# Autodesk Inventor assembly: Full_Assembly_2_0_2
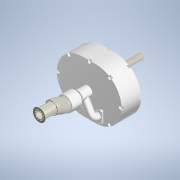
[picture p0: Inventor's stored thumbnail of the model, 180x180]
Saved by Autodesk Inventor 2021 (Build 250183000, 183)
## iProperties
Created: 2021-04-14
Part Number: Full_Assembly_2_0_2
Document SubType Name: Assembly
Designer: lucia
Mass: 12850.4 g
Surface Area: 5748.06 cm^2
Volume: 2623.18 cm^3
Density: 4.89877 g/cm^3
Author: lucia
## Documents named in this file (10)
- E:\Documents\Inventor\Fixed Rotor Wankel Engine\Assemblies\Full_Assembly_2_0_2.iam
- E:\Documents\Inventor\Fixed Rotor Wankel Engine\Parts\Rotor_Mount.ipt
- E:\Documents\Inventor\Fixed Rotor Wankel Engine\Parts\Eccentric_Shaft_2.ipt
- E:\Documents\Inventor\Fixed Rotor Wankel Engine\Parts\Rotor_Geared_6t_Mountable.ipt
- E:\Documents\Inventor\Fixed Rotor Wankel Engine\Parts\Side_Plate_Combined_Intake_Exhaust.ipt
- E:\Documents\Inventor\Fixed Rotor Wankel Engine\Parts\Housing.ipt
- E:\Documents\Inventor\Fixed Rotor Wankel Engine\Parts\Side_Plate_Blank.ipt
- E:\Documents\Inventor\Fixed Rotor Wankel Engine\Parts\Combined_Intake_Exhaust_Manifold.ipt
- E:\Documents\Inventor\Fixed Rotor Wankel Engine\Parts\Intake_Manifold_2.ipt
- E:\Documents\Inventor\Fixed Rotor Wankel Engine\Parts\Exhaust_Manifold_2_2.ipt
## Components (9 placed, 9 different names)
1. Rotor_Mount:1 — Mate:1, Mate:2, Mate:3, Mate:4, Mate:5, Mate:6, Mate:7
2. Eccentric_Shaft_2:1 — Mate:3, Mate:4, Mate:9, Mate:16, Mate:17, Mate:18, Mate:Correct_Position, Rotation:1
3. Rotor_Geared_6t_Mountable:1 — Mate:5, Mate:6, Mate:7, Mate:8
4. Side_Plate_Combined_Intake_Exhaust:1 — Mate:8, Mate:9, Mate:10, Mate:11, Mate:12, Mate:Correct_Position_2, Rotation:1, Mate:27, Mate:28, Mate:26, Mate:29, Mate:30, Mate:31
5. Housing:1 — Mate:10, Mate:11, Mate:12, Mate:13, Mate:14, Mate:15
6. Side_Plate_Blank:1 — Mate:13, Mate:14, Mate:15
7. Combined_Intake_Exhaust_Manifold:1 — Mate:16, Mate:17, Mate:18
8. Intake_Manifold_2:1 — Mate:27, Mate:28, Mate:26
9. Exhaust_Manifold_2_2:1 — Mate:29, Mate:30, Mate:31
## Relationships (27: Mate 26, RelateRotation 1)
- Mate:1: Rotor_Mount:1
- Mate:2: Rotor_Mount:1
- Mate:3: Rotor_Mount:1 ↔ Eccentric_Shaft_2:1
- Mate:4: Rotor_Mount:1 ↔ Eccentric_Shaft_2:1
- Mate:5: Rotor_Mount:1 ↔ Rotor_Geared_6t_Mountable:1
- Mate:6: Rotor_Mount:1 ↔ Rotor_Geared_6t_Mountable:1
- Mate:7: Rotor_Mount:1 ↔ Rotor_Geared_6t_Mountable:1
- Mate:8: Rotor_Geared_6t_Mountable:1 ↔ Side_Plate_Combined_Intake_Exhaust:1
- Mate:9: Eccentric_Shaft_2:1 ↔ Side_Plate_Combined_Intake_Exhaust:1
- Mate:10: Side_Plate_Combined_Intake_Exhaust:1 ↔ Housing:1
- Mate:11: Side_Plate_Combined_Intake_Exhaust:1 ↔ Housing:1
- Mate:12: Side_Plate_Combined_Intake_Exhaust:1 ↔ Housing:1
- Mate:13: Housing:1 ↔ Side_Plate_Blank:1
- Mate:14: Housing:1 ↔ Side_Plate_Blank:1
- Mate:15: Housing:1 ↔ Side_Plate_Blank:1
- Mate:16: Eccentric_Shaft_2:1 ↔ Combined_Intake_Exhaust_Manifold:1
- Mate:17: Eccentric_Shaft_2:1 ↔ Combined_Intake_Exhaust_Manifold:1
- Mate:18: Eccentric_Shaft_2:1 ↔ Combined_Intake_Exhaust_Manifold:1
- Mate:Correct_Position: Eccentric_Shaft_2:1
- Mate:Correct_Position_2: Side_Plate_Combined_Intake_Exhaust:1
- Rotation:1 [RelateRotation] (0.5 ul): Eccentric_Shaft_2:1 ↔ Side_Plate_Combined_Intake_Exhaust:1
- Mate:27: Side_Plate_Combined_Intake_Exhaust:1 ↔ Intake_Manifold_2:1
- Mate:28: Side_Plate_Combined_Intake_Exhaust:1 ↔ Intake_Manifold_2:1
- Mate:26: Side_Plate_Combined_Intake_Exhaust:1 ↔ Intake_Manifold_2:1
- Mate:29: Side_Plate_Combined_Intake_Exhaust:1 ↔ Exhaust_Manifold_2_2:1
- Mate:30: Side_Plate_Combined_Intake_Exhaust:1 ↔ Exhaust_Manifold_2_2:1
- Mate:31: Side_Plate_Combined_Intake_Exhaust:1 ↔ Exhaust_Manifold_2_2:1
